# Autodesk Inventor assembly: Left Wheel
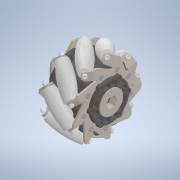
[picture p0: Inventor's stored thumbnail of the model, 180x180]
Saved by Autodesk Inventor 2020 (Build 240168000, 168)
## iProperties
Created: 2022-10-15
Part Number: Left Wheel
Document SubType Name: Assembly
Designer: Jason
Author: Jason
## Documents named in this file (3)
- C:\Users\Jason\Documents\Inventor\FTC Robot 2023\Left Wheel.iam
- C:\Users\Jason\Documents\Inventor\FTC Robot 2023\Left Wheel.ipt
- C:\Users\Jason\Documents\Inventor\FTC Robot 2023\Wheel Bearing.ipt
## Components (3 placed, 2 different names)
1. Left Wheel:1 — Mate:1, Mate:2, Mate:3, Mate:4, Mate:5
2. Wheel Bearing:1 — Mate:1, Mate:2, Mate:3
3. Wheel Bearing:2 — Mate:4, Mate:5
## Relationships (5: Mate 5)
- Mate:1: Left Wheel:1 ↔ Wheel Bearing:1
- Mate:2: Left Wheel:1 ↔ Wheel Bearing:1
- Mate:3: Left Wheel:1 ↔ Wheel Bearing:1
- Mate:4: Left Wheel:1 ↔ Wheel Bearing:2
- Mate:5: Left Wheel:1 ↔ Wheel Bearing:2
